# Autodesk Inventor assembly: frame
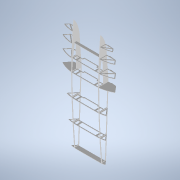
[picture p0: Inventor's stored thumbnail of the model, 180x180]
Saved by Autodesk Inventor 2020.3 (Build 243373010, 373A)
## iProperties
Created: 2020-05-22
Part Number: frame
Document SubType Name: Assembly
Designer: kardo
Mass: 65.1141 g
Surface Area: 856.356 cm^2
Volume: 65.1141 cm^3
Density: 1 g/cm^3
Author: kardo
## Documents named in this file (9)
- D:\Computer Aided Design\hydroplane plan\frame.iam
- D:\Computer Aided Design\hydroplane plan\frame\stringer.ipt
- D:\Computer Aided Design\hydroplane plan\frame\bulkhead_main.ipt
- D:\Computer Aided Design\hydroplane plan\frame\bulkhead_F1.ipt
- D:\Computer Aided Design\hydroplane plan\frame\bulkhead_front.ipt
- D:\Computer Aided Design\hydroplane plan\frame\bulkhead_F2.ipt
- D:\Computer Aided Design\hydroplane plan\frame\bulkhead_B1.ipt
- D:\Computer Aided Design\hydroplane plan\frame\bulkhead_B2.ipt
- D:\Computer Aided Design\hydroplane plan\frame\transom.ipt
## Components (10 placed, 8 different names)
1. stringer:1 — Mate:5, Mate:6, Mate:7, Mate:16, Mate:17, Mate:19
2. stringer:2 — Mate:1, Mate:2, Mate:3, Mate:20, Mate:21, Mate:22, Mate:23, Mate:24, Mate:26, Mate:27, Mate:28, Mate:29, Mate:30, Mate:31, Mate:32, Mate:33, Mate:34, Mate:35, Mate:36, Mate:37, Mate:38
3. bulkhead_main:1 — Mate:1, Mate:2, Mate:3, Mate:5, Mate:6, Mate:7
4. bulkhead_F1:1 — Mate:23, Mate:27, Mate:28
5. bulkhead_front:1 — Mate:24, Mate:26, Mate:29
6. bulkhead_F2:1 — Mate:20, Mate:21, Mate:22
7. bulkhead_F2:2 — Mate:16, Mate:17, Mate:19
8. bulkhead_B1:1 — Mate:30, Mate:31, Mate:32
9. bulkhead_B2:1 — Mate:33, Mate:34, Mate:35
10. transom:1 — Mate:36, Mate:37, Mate:38
## Relationships (27: Mate 27)
- Mate:1: stringer:2 ↔ bulkhead_main:1
- Mate:2: stringer:2 ↔ bulkhead_main:1
- Mate:3: stringer:2 ↔ bulkhead_main:1
- Mate:5: stringer:1 ↔ bulkhead_main:1
- Mate:6: stringer:1 ↔ bulkhead_main:1
- Mate:7: stringer:1 ↔ bulkhead_main:1
- Mate:16: stringer:1 ↔ bulkhead_F2:2
- Mate:17: stringer:1 ↔ bulkhead_F2:2
- Mate:19: stringer:1 ↔ bulkhead_F2:2
- Mate:20: stringer:2 ↔ bulkhead_F2:1
- Mate:21: stringer:2 ↔ bulkhead_F2:1
- Mate:22: stringer:2 ↔ bulkhead_F2:1
- Mate:23: stringer:2 ↔ bulkhead_F1:1
- Mate:24: stringer:2 ↔ bulkhead_front:1
- Mate:26: stringer:2 ↔ bulkhead_front:1
- Mate:27: stringer:2 ↔ bulkhead_F1:1
- Mate:28: stringer:2 ↔ bulkhead_F1:1
- Mate:29: stringer:2 ↔ bulkhead_front:1
- Mate:30: stringer:2 ↔ bulkhead_B1:1
- Mate:31: stringer:2 ↔ bulkhead_B1:1
- Mate:32: stringer:2 ↔ bulkhead_B1:1
- Mate:33: stringer:2 ↔ bulkhead_B2:1
- Mate:34: stringer:2 ↔ bulkhead_B2:1
- Mate:35: stringer:2 ↔ bulkhead_B2:1
- Mate:36: stringer:2 ↔ transom:1
- Mate:37: stringer:2 ↔ transom:1
- Mate:38: stringer:2 ↔ transom:1
